# Autodesk Inventor assembly: tr2
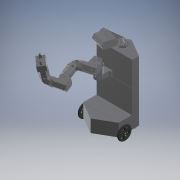
[picture p0: Inventor's stored thumbnail of the model, 180x180]
Saved by Autodesk Inventor 2017 (Build 210142000, 142)
## iProperties
Created: 2018-10-17
Part Number: tr2
Document SubType Name: Assembly
Designer: Administrator
Author: Administrator
## Documents named in this file (5)
- C:\Users\Dell\Documents\GitHub\tr2\TR2.iam
- C:\Users\Dell\Documents\GitHub\tr2\Base\Base.iam
- C:\Users\Dell\Documents\GitHub\tr2\Body\Body.iam
- C:\Users\Dell\Documents\GitHub\tr2\Arm\Arm.iam
- C:\Users\Dell\Documents\GitHub\tr2\Head\Head.iam
## Components (4 placed, 4 different names)
1. Base:1 [sub-assembly] — Mate:2, Mate:27, Mate:28, Mate:29, Mate:30
2. Body:1 [sub-assembly] — Mate:22, Mate:23, Mate:27, Mate:28, Mate:29, Mate:30, Mate:31, Mate:32
3. Arm:1 [sub-assembly] — Mate:22, Mate:31, Mate:32
4. Head:1 [sub-assembly] — Mate:23
## Relationships (9: Mate 9)
- Mate:2 (50 mm): Base:1
- Mate:22: Body:1 ↔ Arm:1
- Mate:23: Body:1 ↔ Head:1
- Mate:27: Base:1 ↔ Body:1
- Mate:28: Base:1 ↔ Body:1
- Mate:29: Base:1 ↔ Body:1
- Mate:30: Base:1 ↔ Body:1
- Mate:31: Body:1 ↔ Arm:1
- Mate:32: Body:1 ↔ Arm:1
